# Autodesk Inventor assembly: VersaPlanetary v2 NoStage
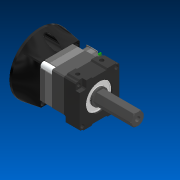
[picture p0: Inventor's stored thumbnail of the model, 180x180]
Saved by Autodesk Inventor 2022.2 (Build 262287000, 287)
## iProperties
Created: 2016-10-31
Part Number: VersaPlanetary v2 NoStage
Description: STEP AP214
Document SubType Name: Assembly
Designer: omard
Mass: 147.211 g
Surface Area: 697.563 cm^2
Volume: 83.5114 cm^3
Density: 1.76276 g/cm^3
Sending System: SolidWorks 2016
Preprocessor: SwSTEP 2.0
Title: 217-4973_2stage_BAG.STEP
Revision Number: ANY
## Documents named in this file (10)
- D:\omard\OneDrive - Auburn University\BasketBall Shooting Robot\VEX Parts\VersaPlanetary v2 NoStage.iam
- D:\omard\OneDrive - Auburn University\BasketBall Shooting Robot\VEX Parts\Components\217-2625-026 Rev1.ipt
- D:\omard\OneDrive - Auburn University\BasketBall Shooting Robot\VEX Parts\Components\217-2742-001 Rev4.ipt
- D:\omard\OneDrive - Auburn University\BasketBall Shooting Robot\VEX Parts\Components\217-2625-017 Rev1_9714K61.ipt
- D:\omard\OneDrive - Auburn University\BasketBall Shooting Robot\VEX Parts\Components\217-2625-003 Rev1.ipt
- D:\omard\OneDrive - Auburn University\BasketBall Shooting Robot\VEX Parts\Components\217-2625-018 Rev1_98541A410.ipt
- D:\omard\OneDrive - Auburn University\BasketBall Shooting Robot\VEX Parts\Components\217-2820 Rev1_Public.iam
- D:\omard\OneDrive - Auburn University\BasketBall Shooting Robot\VEX Parts\Components\217-2816-001 Rev1.ipt
- D:\omard\OneDrive - Auburn University\BasketBall Shooting Robot\VEX Parts\VersaPlanetary Integrated Encoder (217-5046).iam
- D:\omard\OneDrive - Auburn University\BasketBall Shooting Robot\VEX Parts\VersaPlanetary CIM Adapter (217-4018).ipt
## Components (10 placed, 10 different names)
1. 217-2625-026 Rev1_1 — Angle:1, Mate:5, Mate:6, Angle:2, Mate:7, Mate:10, Mate:11, Mate:12, Angle:3
2. 217-2742-001 Rev4_2
3. 217-2742-001 Rev4_3 — Mate:3, Mate:4, Mate:5, Mate:6, Angle:2
4. 217-2625-017 Rev1_9714K61_4
5. 217-2625-003 Rev1_5 — Mate:3, Mate:4, Angle:1, Mate:8, Angle:3
6. 217-2625-018 Rev1_98541A410_6
7. 217-2820 Rev1_Public_16 [sub-assembly] — Mate:7, Mate:8
8. 217-2816-001 Rev1_17 — Mate:1, Mate:2, Mate:9, Mate:10, Mate:11, Mate:12
9. VersaPlanetary Integrated Encoder (217-5046):1 [sub-assembly] — Mate:1, Mate:2, Mate:9, Mate:13, Mate:14, Mate:15
10. VersaPlanetary CIM Adapter (217-4018):1 — Mate:13, Mate:14, Mate:15
## Relationships (18: Mate 15, Angle 3)
- Mate:1: 217-2816-001 Rev1_17 ↔ VersaPlanetary Integrated Encoder (217-5046):1
- Mate:2: 217-2816-001 Rev1_17 ↔ VersaPlanetary Integrated Encoder (217-5046):1
- Mate:3: 217-2742-001 Rev4_3 ↔ 217-2625-003 Rev1_5
- Mate:4: 217-2742-001 Rev4_3 ↔ 217-2625-003 Rev1_5
- Angle:1 (0 deg): 217-2625-026 Rev1_1 ↔ 217-2625-003 Rev1_5
- Mate:5: 217-2625-026 Rev1_1 ↔ 217-2742-001 Rev4_3
- Mate:6: 217-2625-026 Rev1_1 ↔ 217-2742-001 Rev4_3
- Angle:2 (0 deg): 217-2625-026 Rev1_1 ↔ 217-2742-001 Rev4_3
- Mate:7: 217-2625-026 Rev1_1 ↔ 217-2820 Rev1_Public_16
- Mate:8: 217-2625-003 Rev1_5 ↔ 217-2820 Rev1_Public_16
- Mate:9: 217-2816-001 Rev1_17 ↔ VersaPlanetary Integrated Encoder (217-5046):1
- Mate:10: 217-2625-026 Rev1_1 ↔ 217-2816-001 Rev1_17
- Mate:11: 217-2625-026 Rev1_1 ↔ 217-2816-001 Rev1_17
- Mate:12: 217-2625-026 Rev1_1 ↔ 217-2816-001 Rev1_17
- Angle:3 (0 deg): 217-2625-026 Rev1_1 ↔ 217-2625-003 Rev1_5
- Mate:13: VersaPlanetary Integrated Encoder (217-5046):1 ↔ VersaPlanetary CIM Adapter (217-4018):1
- Mate:14: VersaPlanetary Integrated Encoder (217-5046):1 ↔ VersaPlanetary CIM Adapter (217-4018):1
- Mate:15: VersaPlanetary Integrated Encoder (217-5046):1 ↔ VersaPlanetary CIM Adapter (217-4018):1
